# Autodesk Inventor assembly: Housing_Assembly
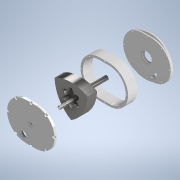
[picture p0: Inventor's stored thumbnail of the model, 180x180]
Saved by Autodesk Inventor 2021 (Build 250183000, 183)
## iProperties
Created: 2021-03-28
Part Number: Housing_Assembly
Document SubType Name: Assembly
Designer: lucia
Author: lucia
## Documents named in this file (7)
- E:\Documents\Inventor\Fixed Rotor Wankel Engine\Assemblies\Housing_Assembly.iam
- E:\Documents\Inventor\Fixed Rotor Wankel Engine\Parts\Rotor_Mount.ipt
- E:\Documents\Inventor\Fixed Rotor Wankel Engine\Parts\Eccentric_Shaft.ipt
- E:\Documents\Inventor\Fixed Rotor Wankel Engine\Parts\Rotor_Geared_6t_Mountable.ipt
- E:\Documents\Inventor\Fixed Rotor Wankel Engine\Parts\Side_Plate_Geared.ipt
- E:\Documents\Inventor\Fixed Rotor Wankel Engine\Parts\Housing.ipt
- E:\Documents\Inventor\Fixed Rotor Wankel Engine\Parts\Side_Plate_Intake_Exhaust.ipt
## Components (6 placed, 6 different names)
1. Rotor_Mount:1 — Mate:1, Flush:1, Mate:3, Mate:4, Mate:5, Mate:6, Mate:7
2. Eccentric_Shaft:1 — Mate:3, Mate:4, Mate:9
3. Rotor_Geared_6t_Mountable:1 — Mate:5, Mate:6, Mate:7, Mate:8
4. Side_Plate_Geared:1 — Mate:8, Mate:9, Mate:10, Mate:11, Mate:12
5. Housing:1 — Mate:10, Mate:11, Mate:12, Mate:13, Mate:14, Mate:15
6. Side_Plate_Intake_Exhaust:1 — Mate:13, Mate:14, Mate:15
## Relationships (16: Mate 15, Flush 1)
- Mate:1: Rotor_Mount:1
- Mate:2
- Flush:1: Rotor_Mount:1
- Mate:3: Rotor_Mount:1 ↔ Eccentric_Shaft:1
- Mate:4: Rotor_Mount:1 ↔ Eccentric_Shaft:1
- Mate:5: Rotor_Mount:1 ↔ Rotor_Geared_6t_Mountable:1
- Mate:6: Rotor_Mount:1 ↔ Rotor_Geared_6t_Mountable:1
- Mate:7: Rotor_Mount:1 ↔ Rotor_Geared_6t_Mountable:1
- Mate:8 (203.2 mm): Rotor_Geared_6t_Mountable:1 ↔ Side_Plate_Geared:1
- Mate:9: Eccentric_Shaft:1 ↔ Side_Plate_Geared:1
- Mate:10 (381 mm): Side_Plate_Geared:1 ↔ Housing:1
- Mate:11: Side_Plate_Geared:1 ↔ Housing:1
- Mate:12: Side_Plate_Geared:1 ↔ Housing:1
- Mate:13 (177.8 mm): Housing:1 ↔ Side_Plate_Intake_Exhaust:1
- Mate:14: Housing:1 ↔ Side_Plate_Intake_Exhaust:1
- Mate:15: Housing:1 ↔ Side_Plate_Intake_Exhaust:1
